# Autodesk Inventor assembly: Lower box main assembly 6
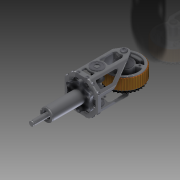
[picture p0: Inventor's stored thumbnail of the model, 180x180]
Saved by Autodesk Inventor 2012 (Build 160160000, 160)
## iProperties
Created: 2013-08-26
Part Number: Lower box main assembly 6
Document SubType Name: Assembly
Designer: Bryce
Author: Bryce
## Documents named in this file (17)
- C:\Users\Bryce\Dropbox\Inventor Design Project Files\Independent Swerves\Inventor 2012\Lower box main assembly 6.iam
- C:\Users\Bryce\Dropbox\Inventor Design Project Files\Independent Swerves\Inventor 2012\lower box upper plate 2.ipt
- C:\Users\Bryce\Dropbox\Inventor Design Project Files\Independent Swerves\Inventor 2012\lower bix side plate 5.ipt
- C:\Users\Bryce\Dropbox\Inventor Design Project Files\Independent Swerves\Inventor 2012\lower box weel shaft steel 2.ipt
- C:\Users\Bryce\Dropbox\Inventor Design Project Files\Independent Swerves\Inventor 2012\wheel 3in custom.ipt
- C:\Users\Bryce\Dropbox\Inventor Design Project Files\Independent Swerves\Imported Components\32t #25 sprocket.ipt
- C:\Users\Bryce\Dropbox\Inventor Design Project Files\Independent Swerves\Inventor 2012\.375 ID .875 OD bearing.ipt
- C:\Users\Bryce\Dropbox\Inventor Design Project Files\Independent Swerves\Inventor 2012\lower box upper shaft.ipt
- C:\Users\Bryce\Dropbox\Inventor Design Project Files\Independent Swerves\Imported Components\12t #25 sprocket.ipt
- C:\Users\Bryce\Dropbox\Inventor Design Project Files\Independent Swerves\Imported Components\miters.ipt
- C:\Users\Bryce\Dropbox\Inventor Design Project Files\Independent Swerves\Inventor 2012\lower box bolt plate.ipt
- C:\Users\Bryce\Dropbox\Inventor Design Project Files\Independent Swerves\Inventor 2012\new wheel rim.ipt
- C:\Users\Bryce\Dropbox\Inventor Design Project Files\Independent Swerves\Inventor 2012\.5 id 1.125 od flange bearing.ipt
- C:\Users\Bryce\Dropbox\Inventor Design Project Files\Independent Swerves\Inventor 2012\6 32 bolt 0.5''.ipt
- C:\Users\Bryce\Dropbox\Inventor Design Project Files\Independent Swerves\Inventor 2012\10 32 bolt 0.75.ipt
- C:\Users\Bryce\Dropbox\Inventor Design Project Files\Independent Swerves\Inventor 2012\turn shaft 3.ipt
- C:\Users\Bryce\Dropbox\Inventor Design Project Files\Independent Swerves\Inventor 2012\vertical drive shaft 4.ipt
## Components (31 placed, 16 different names)
1. lower box upper plate 2:1 — Mate:2, Mate:4, Angle:1, Mate:16, Insert:4, Mate:17, Mate:20, Mate:21, Mate:22, Mate:23
2. lower bix side plate 5:1 — Mate:2, Mate:6, Insert:2, Flush:3, Mate:20, Mate:21, Insert:9, Insert:10, Insert:11, Insert:12, Insert:13, Insert:14
3. lower bix side plate 5:2 — Mate:4, Insert:1, Insert:3, Mate:22, Mate:23, Mate:24, Insert:15, Insert:16, Insert:17, Insert:18, Insert:19, Insert:20
4. lower box weel shaft steel 2:1 — Insert:1, Mate:5, Insert:21, Insert:22
5. wheel 3in custom:1 — Mate:5, Mate:6, Mate:7, Mate:8, Mate:9, Insert:6, Rotation:3, Insert:7, Insert:8
6. 32t #25 sprocket:1 — Mate:7, Mate:8, Mate:9, Flush:4, Mate:12, Mate:14, Rotation:2
7. .375 ID .875 OD bearing:1 — Insert:2, Mate:10
8. .375 ID .875 OD bearing:2 — Insert:3
9. lower box upper shaft:1 — Mate:10, Flush:3, Mate:11, Mate:15, Rotation:1, Flush:6
10. 12t #25 sprocket:1 — Mate:11, Flush:4, Mate:13, Rotation:2, Flush:6
11. miters:1 — Mate:15, Angle:1, Mate:16, Flush:5, Mate:24
12. turn shaft 3:1 — Insert:4, Insert:5, Mate:18, Mate:19
13. lower box bolt plate:1 — Insert:5, Mate:17, Mate:18
14. vertical drive shaft 4:1 — Mate:19, Flush:5, Rotation:1
15. new wheel rim:1 — Insert:6, Rotation:3
16. .5 id 1.125 od flange bearing:1 — Insert:7
17. .5 id 1.125 od flange bearing:2 — Insert:8
18. 6 32 bolt 0.5'':1 — Insert:14
19. 6 32 bolt 0.5'':2 — Insert:13
20. 6 32 bolt 0.5'':3 — Insert:10
21. 6 32 bolt 0.5'':4 — Insert:9
22. 6 32 bolt 0.5'':5 — Insert:12
23. 6 32 bolt 0.5'':6 — Insert:11
24. 6 32 bolt 0.5'':7 — Insert:20
25. 6 32 bolt 0.5'':8 — Insert:19
26. 6 32 bolt 0.5'':9 — Insert:18
27. 6 32 bolt 0.5'':10 — Insert:17
28. 6 32 bolt 0.5'':11 — Insert:16
29. 6 32 bolt 0.5'':12 — Insert:15
30. 10 32 bolt 0.75:1 — Insert:21
31. 10 32 bolt 0.75:2 — Insert:22
## Relationships (52: Mate 22, Insert 22, Flush 4, RelateRotation 3, Angle 1)
- Mate:2: lower box upper plate 2:1 ↔ lower bix side plate 5:1
- Mate:4: lower box upper plate 2:1 ↔ lower bix side plate 5:2
- Insert:1: lower bix side plate 5:2 ↔ lower box weel shaft steel 2:1
- Mate:5: lower box weel shaft steel 2:1 ↔ wheel 3in custom:1
- Mate:6 (19.05 mm): lower bix side plate 5:1 ↔ wheel 3in custom:1
- Mate:7: wheel 3in custom:1 ↔ 32t #25 sprocket:1
- Mate:8: wheel 3in custom:1 ↔ 32t #25 sprocket:1
- Mate:9: wheel 3in custom:1 ↔ 32t #25 sprocket:1
- Insert:2: lower bix side plate 5:1 ↔ .375 ID .875 OD bearing:1
- Insert:3: lower bix side plate 5:2 ↔ .375 ID .875 OD bearing:2
- Mate:10: .375 ID .875 OD bearing:1 ↔ lower box upper shaft:1
- Flush:3: lower bix side plate 5:1 ↔ lower box upper shaft:1
- Mate:11: lower box upper shaft:1 ↔ 12t #25 sprocket:1
- Flush:4: 32t #25 sprocket:1 ↔ 12t #25 sprocket:1
- Mate:12: 32t #25 sprocket:1
- Mate:13: 12t #25 sprocket:1
- Mate:14: 32t #25 sprocket:1
- Mate:15: lower box upper shaft:1 ↔ miters:1
- Angle:1 (0 deg): lower box upper plate 2:1 ↔ miters:1
- Mate:16 (-31.75 mm): lower box upper plate 2:1 ↔ miters:1
- Insert:4: lower box upper plate 2:1 ↔ turn shaft 3:1
- Insert:5: turn shaft 3:1 ↔ lower box bolt plate:1
- Mate:17 (0.0127 mm): lower box upper plate 2:1 ↔ lower box bolt plate:1
- Mate:18: turn shaft 3:1 ↔ lower box bolt plate:1
- Mate:19: turn shaft 3:1 ↔ vertical drive shaft 4:1
- Flush:5: miters:1 ↔ vertical drive shaft 4:1
- Rotation:1 [RelateRotation] (1 ul): lower box upper shaft:1 ↔ vertical drive shaft 4:1
- Rotation:2 [RelateRotation] (0.3333 ul): 32t #25 sprocket:1 ↔ 12t #25 sprocket:1
- Flush:6: lower box upper shaft:1 ↔ 12t #25 sprocket:1
- Insert:6: wheel 3in custom:1 ↔ new wheel rim:1
- Rotation:3 [RelateRotation] (1 ul): wheel 3in custom:1 ↔ new wheel rim:1
- Insert:7: wheel 3in custom:1 ↔ .5 id 1.125 od flange bearing:1
- Insert:8: wheel 3in custom:1 ↔ .5 id 1.125 od flange bearing:2
- Mate:20: lower box upper plate 2:1 ↔ lower bix side plate 5:1
- Mate:21: lower box upper plate 2:1 ↔ lower bix side plate 5:1
- Mate:22: lower box upper plate 2:1 ↔ lower bix side plate 5:2
- Mate:23: lower box upper plate 2:1 ↔ lower bix side plate 5:2
- Mate:24 (6.35 mm): lower bix side plate 5:2 ↔ miters:1
- Insert:9: lower bix side plate 5:1 ↔ 6 32 bolt 0.5'':4
- Insert:10: lower bix side plate 5:1 ↔ 6 32 bolt 0.5'':3
- Insert:11: lower bix side plate 5:1 ↔ 6 32 bolt 0.5'':6
- Insert:12: lower bix side plate 5:1 ↔ 6 32 bolt 0.5'':5
- Insert:13: lower bix side plate 5:1 ↔ 6 32 bolt 0.5'':2
- Insert:14: lower bix side plate 5:1 ↔ 6 32 bolt 0.5'':1
- Insert:15: lower bix side plate 5:2 ↔ 6 32 bolt 0.5'':12
- Insert:16: lower bix side plate 5:2 ↔ 6 32 bolt 0.5'':11
- Insert:17: lower bix side plate 5:2 ↔ 6 32 bolt 0.5'':10
- Insert:18: lower bix side plate 5:2 ↔ 6 32 bolt 0.5'':9
- Insert:19: lower bix side plate 5:2 ↔ 6 32 bolt 0.5'':8
- Insert:20: lower bix side plate 5:2 ↔ 6 32 bolt 0.5'':7
- Insert:21: lower box weel shaft steel 2:1 ↔ 10 32 bolt 0.75:1
- Insert:22: lower box weel shaft steel 2:1 ↔ 10 32 bolt 0.75:2
